# Autodesk Inventor assembly: Base
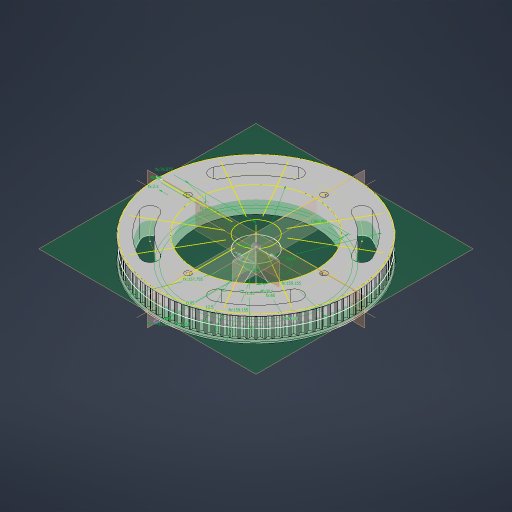
[picture p0: Inventor's stored thumbnail of the model, 512x512]
Saved by Autodesk Inventor 2024 (Build 280153000, 153)
## iProperties
Created: 2023-10-21
Part Number: Base
Document SubType Name: Assembly
Designer: range
Author: range
## Documents named in this file (3)
- C:\Users\range\CodingProjects\C-AAM\CAD\V1\Base.iam
- C:\Users\range\CodingProjects\C-AAM\CAD\V1\Parts\LazySusan.iam
- C:\Users\range\CodingProjects\C-AAM\CAD\V1\LargePitchAssembly.iam
## Components (2 placed, 2 different names)
1. LazySusan:1 [sub-assembly]
2. LargePitchAssembly:1 [sub-assembly]
## Relationships (2: Mate 2)
- [Mate] (2.5 mm): LazySusan:1 ↔ LargePitchAssembly:1
- [Mate]: LazySusan:1 ↔ LargePitchAssembly:1
